# Autodesk Inventor assembly: Lift2
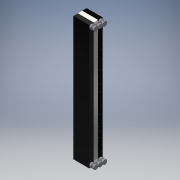
[picture p0: Inventor's stored thumbnail of the model, 180x180]
Saved by Autodesk Inventor 2017 (Build 210142000, 142)
## iProperties
Created: 2017-02-01
Part Number: Lift2
Document SubType Name: Assembly
Designer: RoboticsUser
Author: RoboticsUser
## Documents named in this file (3)
- C:\Robotics\CAD\2016-17_CAD\Lift2.iam
- C:\Robotics\CAD\2016-17_CAD\LiftSlidePart.ipt
- C:\Robotics\CAD\2016-17_CAD\LiftPully.ipt
## Components (9 placed, 2 different names)
1. LiftSlidePart:2 — Mate:2, Tangent:3, Tangent:4, Mate:6, Flush:3, Flush:4, Mate:8, Tangent:9, Tangent:14, Mate:12
2. LiftSlidePart:3 — Mate:3, Tangent:5, Tangent:6, Mate:6, Flush:3, Flush:4, Mate:7, Flush:5, Flush:6, Mate:10, Tangent:13
3. LiftSlidePart:4 — Mate:4, Tangent:7, Tangent:8, Mate:7, Flush:5, Flush:6, Mate:11, Tangent:15, Tangent:16
4. LiftPully:1 — Mate:2, Tangent:3, Tangent:4
5. LiftPully:2 — Mate:3, Tangent:5, Tangent:6
6. LiftPully:4 — Mate:4, Tangent:7, Tangent:8
7. LiftPully:5 — Mate:10, Tangent:13, Tangent:14
8. LiftPully:6 — Mate:11, Tangent:15, Tangent:16
9. LiftPully:8 — Mate:8, Tangent:9, Mate:12
## Relationships (24: Tangent 11, Mate 9, Flush 4)
- Mate:2: LiftSlidePart:2 ↔ LiftPully:1
- Tangent:3: LiftSlidePart:2 ↔ LiftPully:1
- Tangent:4: LiftSlidePart:2 ↔ LiftPully:1
- Mate:3: LiftSlidePart:3 ↔ LiftPully:2
- Tangent:5: LiftSlidePart:3 ↔ LiftPully:2
- Tangent:6: LiftSlidePart:3 ↔ LiftPully:2
- Mate:4: LiftSlidePart:4 ↔ LiftPully:4
- Tangent:7: LiftSlidePart:4 ↔ LiftPully:4
- Tangent:8: LiftSlidePart:4 ↔ LiftPully:4
- Mate:6: LiftSlidePart:2 ↔ LiftSlidePart:3
- Flush:3: LiftSlidePart:2 ↔ LiftSlidePart:3
- Flush:4: LiftSlidePart:2 ↔ LiftSlidePart:3
- Mate:7: LiftSlidePart:3 ↔ LiftSlidePart:4
- Flush:5: LiftSlidePart:3 ↔ LiftSlidePart:4
- Flush:6: LiftSlidePart:3 ↔ LiftSlidePart:4
- Mate:8: LiftSlidePart:2 ↔ LiftPully:8
- Tangent:9: LiftSlidePart:2 ↔ LiftPully:8
- Mate:10: LiftSlidePart:3 ↔ LiftPully:5
- Tangent:13: LiftSlidePart:3 ↔ LiftPully:5
- Tangent:14: LiftSlidePart:2 ↔ LiftPully:5
- Mate:11: LiftSlidePart:4 ↔ LiftPully:6
- Tangent:15: LiftSlidePart:4 ↔ LiftPully:6
- Tangent:16: LiftSlidePart:4 ↔ LiftPully:6
- Mate:12 (-6.35 mm): LiftSlidePart:2 ↔ LiftPully:8
